# Autodesk Inventor assembly: Assembly1
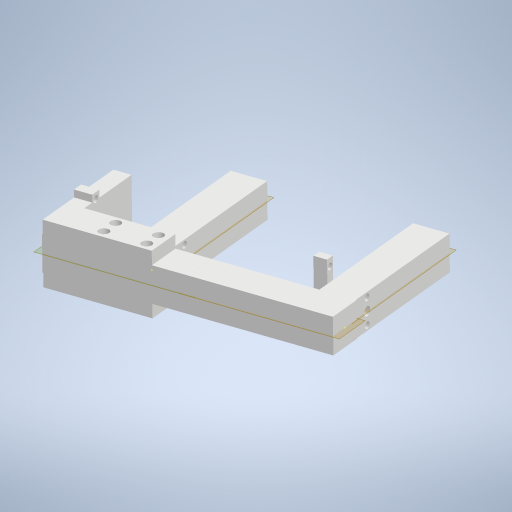
[picture p0: Inventor's stored thumbnail of the model, 512x512]
Saved by Autodesk Inventor 2024 (Build 280153000, 153)
## iProperties
Created: 2024-01-10
Part Number: Assembly1
Document SubType Name: Assembly
Designer: aidan
Author: aidan
## Documents named in this file (5)
- C:\Users\aidan\OneDrive\Documents\Inventor\Content Center Files\Assembly1.iam
- C:\Users\aidan\OneDrive\Documents\Inventor\Content Center Files\1in square tube.ipt
- C:\Users\aidan\OneDrive\Documents\Inventor\Content Center Files\Lead Nut Holder.ipt
- C:\Users\aidan\OneDrive\Documents\Inventor\Content Center Files\1in square tube with holes.ipt
- C:\Users\aidan\OneDrive\Documents\Inventor\Content Center Files\Motor Mount.ipt
## Components (6 placed, 4 different names)
1. 1in square tube:1 — Mate:3, Mate:4, Mate:5
2. Lead Nut Holder:1 — Mate:3, Mate:4
3. 1in square tube with holes:1 — Mate:5, Mate:6, Mate:7, Mate:8
4. 1in square tube with holes:2 — Mate:6, Mate:7, Mate:8, Mate:9, Mate:10, Mate:11, Mate:12
5. Motor Mount:1 — Mate:9, Mate:10
6. 1in square tube:2 — Mate:11, Mate:12
## Relationships (10: Mate 10)
- Mate:3: 1in square tube:1 ↔ Lead Nut Holder:1
- Mate:4: 1in square tube:1 ↔ Lead Nut Holder:1
- Mate:5: 1in square tube:1 ↔ 1in square tube with holes:1
- Mate:6: 1in square tube with holes:1 ↔ 1in square tube with holes:2
- Mate:7: 1in square tube with holes:1 ↔ 1in square tube with holes:2
- Mate:8: 1in square tube with holes:1 ↔ 1in square tube with holes:2
- Mate:9: 1in square tube with holes:2 ↔ Motor Mount:1
- Mate:10: 1in square tube with holes:2 ↔ Motor Mount:1
- Mate:11: 1in square tube with holes:2 ↔ 1in square tube:2
- Mate:12: 1in square tube with holes:2 ↔ 1in square tube:2
